# Autodesk Inventor assembly: Application_smartphone_microscope_v3
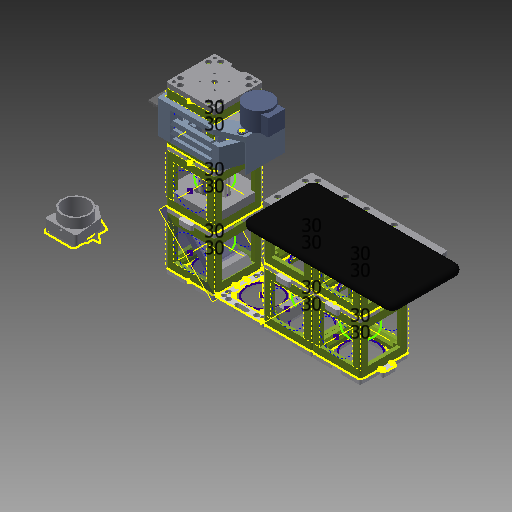
[picture p0: Inventor's stored thumbnail of the model, 512x512]
Saved by Autodesk Inventor 2019 (Build 230136000, 136)
## iProperties
Created: 2019-07-16
Part Number: Application_smartphone_microscope_v3
Document SubType Name: Assembly
Designer: marsikovabarbora
Author: marsikovabarbora
## Documents named in this file (7)
- C:\Users\marsikovabarbora\Dropbox\UC2\02_CAD\INVENTOR\uc2_v3\Application_smartphone_microscope_Zsample_v3.iam
- C:\Users\marsikovabarbora\Dropbox\UC2\02_CAD\INVENTOR\uc2_v3\Assembly_Cube_empty_IM_v3.iam
- C:\Users\marsikovabarbora\Dropbox\UC2\02_CAD\INVENTOR\uc2_v3\Assembly_Cube_Eyepiece_v3.iam
- C:\Users\marsikovabarbora\Dropbox\UC2\02_CAD\INVENTOR\uc2_v3\Assembly_Cube_Mirror_30x30_v3.iam
- C:\Users\marsikovabarbora\Dropbox\UC2\02_CAD\INVENTOR\uc2_v3\00_Huawei_P20.ipt
- C:\Users\marsikovabarbora\Dropbox\UC2\02_CAD\INVENTOR\uc2_v3\10_Base_puzzle_v3.ipt
- C:\Users\marsikovabarbora\Dropbox\UC2\02_CAD\INVENTOR\uc2_v3\Assembly_Cube_Z-Focus_Sample_v3.iam
## Components (14 placed, 6 different names)
1. Assembly_Cube_Mirror_30x30_v3:1 [sub-assembly] — Mate:39
2. Assembly_Cube_Mirror_30x30_v3:2 [sub-assembly] — Mate:40, Angle:3, Mate:44, Mate:45
3. Assembly_Cube_empty_IM_v3:3 [sub-assembly] — Mate:34, Mate:36, Angle:7, Mate:47
4. Assembly_Cube_empty_IM_v3:5 [sub-assembly] — Mate:37, Mate:43, Angle:6
5. Assembly_Cube_Eyepiece_v3:1 [sub-assembly] — Passend:26, Passend:27, Mate:41, Angle:4, Mate:42
6. 00_Huawei_P20:1 — Passend:26, Passend:27
7. Assembly_Cube_Z-Focus_Sample_v3:1 [sub-assembly] — Mate:38, Angle:2
8. 10_Base_puzzle_v3:1 — Mate:31, Mate:32, Flush:5, Mate:34, Mate:43, Angle:6
9. 10_Base_puzzle_v3:3 — Mate:40, Angle:3, Mate:45
10. 10_Base_puzzle_v3:4
11. 10_Base_puzzle_v3:5 — Angle:1, Mate:39
12. 10_Base_puzzle_v3:2 — Mate:36, Mate:37, Angle:7, Mate:47
13. 10_Base_puzzle_v3:6 — Mate:41, Angle:4, Mate:42, Mate:44
14. 10_Base_puzzle_v3:8 — Mate:38, Angle:1, Angle:2
## Component patterns: (4 elements, first: 10_Base_puzzle_v3:1), (4 elements, first: 10_Base_puzzle_v3:2)
## Relationships (23: Mate 16, Angle 6, Flush 1)
- Passend:26 [Mate]: Assembly_Cube_Eyepiece_v3:1 ↔ 00_Huawei_P20:1
- Passend:27 [Mate]: Assembly_Cube_Eyepiece_v3:1 ↔ 00_Huawei_P20:1
- Mate:31: 10_Base_puzzle_v3:1
- Mate:32: 10_Base_puzzle_v3:1
- Flush:5: 10_Base_puzzle_v3:1
- Mate:34: Assembly_Cube_empty_IM_v3:3 ↔ 10_Base_puzzle_v3:1
- Mate:36: Assembly_Cube_empty_IM_v3:3 ↔ 10_Base_puzzle_v3:2
- Mate:37: Assembly_Cube_empty_IM_v3:5 ↔ 10_Base_puzzle_v3:2
- Mate:38: Assembly_Cube_Z-Focus_Sample_v3:1 ↔ 10_Base_puzzle_v3:8
- Angle:1 (0 deg): 10_Base_puzzle_v3:5 ↔ 10_Base_puzzle_v3:8
- Angle:2 (0 deg): Assembly_Cube_Z-Focus_Sample_v3:1 ↔ 10_Base_puzzle_v3:8
- Mate:39: Assembly_Cube_Mirror_30x30_v3:1 ↔ 10_Base_puzzle_v3:5
- Mate:40: Assembly_Cube_Mirror_30x30_v3:2 ↔ 10_Base_puzzle_v3:3
- Mate:41: Assembly_Cube_Eyepiece_v3:1 ↔ 10_Base_puzzle_v3:6
- Angle:3 (0 deg): Assembly_Cube_Mirror_30x30_v3:2 ↔ 10_Base_puzzle_v3:3
- Angle:4 (0 deg): Assembly_Cube_Eyepiece_v3:1 ↔ 10_Base_puzzle_v3:6
- Mate:42: Assembly_Cube_Eyepiece_v3:1 ↔ 10_Base_puzzle_v3:6
- Mate:43: Assembly_Cube_empty_IM_v3:5 ↔ 10_Base_puzzle_v3:1
- Mate:44: Assembly_Cube_Mirror_30x30_v3:2 ↔ 10_Base_puzzle_v3:6
- Mate:45: Assembly_Cube_Mirror_30x30_v3:2 ↔ 10_Base_puzzle_v3:3
- Angle:6 (0 deg): Assembly_Cube_empty_IM_v3:5 ↔ 10_Base_puzzle_v3:1
- Angle:7 (0 deg): Assembly_Cube_empty_IM_v3:3 ↔ 10_Base_puzzle_v3:2
- Mate:47: Assembly_Cube_empty_IM_v3:3 ↔ 10_Base_puzzle_v3:2
